# Autodesk Inventor assembly: Matrix_12-0056
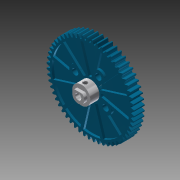
[picture p0: Inventor's stored thumbnail of the model, 180x180]
Saved by Autodesk Inventor 2015 SP1 (Build 190203100, 203)
## iProperties
Category: Gear Kit
Company: Autodesk Inc.
Created: 2014-11-29
Part Number: Matrix_12-0056
Document SubType Name: Assembly
Designer: Matrix
Catalog Web Link: http://matrixrobotics.com/
Vendor: Matrix
Author: Autodesk Inc.
## Documents named in this file (3)
- D:\Data Folder\FTC 2015\KOP\Matrix\Matrix_12-0056.iam
- D:\Data Folder\FTC 2015\KOP\Matrix\Matrix_12-0056_Gear.ipt
- D:\Data Folder\FTC 2015\KOP\Matrix\Matrix_12-0056_Insert.ipt
## Components (2 placed, 2 different names)
1. Matrix_12-0056_Gear:1 — Insert:1
2. Matrix_12-0056_Insert:1 — Insert:1, Angle:1
## Relationships (2: Insert 1, Angle 1)
- Insert:1 (-0.5 mm): Matrix_12-0056_Gear:1 ↔ Matrix_12-0056_Insert:1
- Angle:1 (0 deg): Matrix_12-0056_Insert:1
